# Autodesk Inventor assembly: RearGearboxAssembly
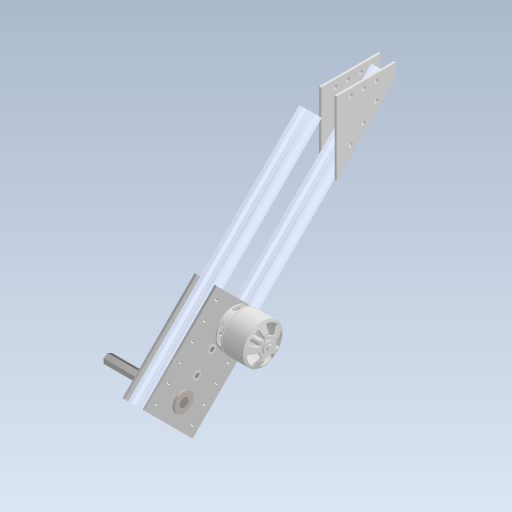
[picture p0: Inventor's stored thumbnail of the model, 512x512]
Saved by Autodesk Inventor 2023 (Build 270158000, 158)
## iProperties
Created: 2023-02-14
Part Number: RearGearboxAssembly
Document SubType Name: Assembly
Designer: Dave
Author: Dave
## Documents named in this file (5)
- C:\Users\Dave\Documents\GitHub\BehrendURCMechanical\CAD\Chassis\GearBox\Final Gears\RearGearboxAssembly.iam
- C:\Users\Dave\Documents\GitHub\BehrendURCMechanical\CAD\Chassis\GearBox\Final Gears\Gearbox Assembly.iam
- C:\Users\Dave\Documents\GitHub\BehrendURCMechanical\CAD\Chassis\20 Profile\CH-1-01-20 Channel 0.362m.ipt
- C:\Users\Dave\Documents\GitHub\BehrendURCMechanical\CAD\Chassis\20 Profile\CH-1-01-20 Channel 0.438m.ipt
- C:\Users\Dave\Documents\GitHub\BehrendURCMechanical\CAD\Chassis\CH-1-01-FrontKneeJoint.ipt
## Components (5 placed, 4 different names)
1. Gearbox Assembly:1 [sub-assembly] — Angle:1, Flush:1, Flush:3, Mate:1
2. CH-1-01-20 Channel 0.362m:1 — Flush:1, Flush:2, Flush:4, Flush:5
3. CH-1-01-20 Channel 0.438m:1 — Flush:2, Flush:3, Mate:1, Flush:4, Flush:5, Flush:6, Mate:2, Mate:3, Mate:4
4. CH-1-01-FrontKneeJoint:1 — Flush:6, Mate:2, Flush:7, Flush:8, Mate:4
5. CH-1-01-FrontKneeJoint:2 — Mate:3, Flush:7, Flush:8
## Relationships (13: Flush 8, Mate 4, Angle 1)
- Angle:1 (45 deg): Gearbox Assembly:1
- Flush:1: Gearbox Assembly:1 ↔ CH-1-01-20 Channel 0.362m:1
- Flush:2: CH-1-01-20 Channel 0.362m:1 ↔ CH-1-01-20 Channel 0.438m:1
- Flush:3 (2.9718 mm): Gearbox Assembly:1 ↔ CH-1-01-20 Channel 0.438m:1
- Mate:1 (3.32 mm): Gearbox Assembly:1 ↔ CH-1-01-20 Channel 0.438m:1
- Flush:4: CH-1-01-20 Channel 0.362m:1 ↔ CH-1-01-20 Channel 0.438m:1
- Flush:5 (-76.2 mm): CH-1-01-20 Channel 0.362m:1 ↔ CH-1-01-20 Channel 0.438m:1
- Flush:6: CH-1-01-20 Channel 0.438m:1 ↔ CH-1-01-FrontKneeJoint:1
- Mate:2: CH-1-01-20 Channel 0.438m:1 ↔ CH-1-01-FrontKneeJoint:1
- Mate:3: CH-1-01-20 Channel 0.438m:1 ↔ CH-1-01-FrontKneeJoint:2
- Flush:7: CH-1-01-FrontKneeJoint:1 ↔ CH-1-01-FrontKneeJoint:2
- Flush:8: CH-1-01-FrontKneeJoint:1 ↔ CH-1-01-FrontKneeJoint:2
- Mate:4: CH-1-01-20 Channel 0.438m:1 ↔ CH-1-01-FrontKneeJoint:1
